# Autodesk Inventor assembly: XY Joint Left (Tulip)
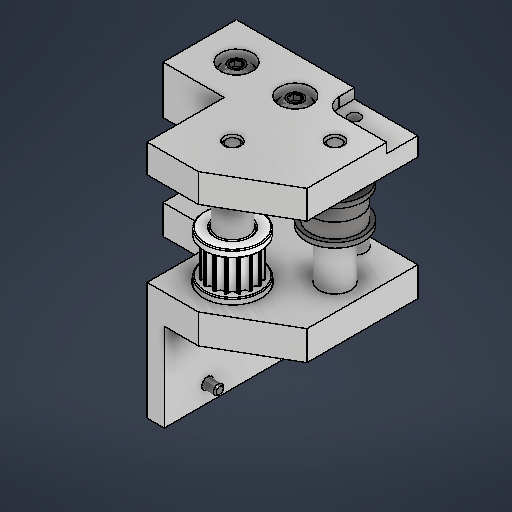
[picture p0: Inventor's stored thumbnail of the model, 512x512]
Saved by Autodesk Inventor 2026 (Build 300175050, 175E)
## iProperties
Created: 2025-05-24
Part Number: XY Joint Left (Tulip)
Document SubType Name: Assembly
Designer: Joshua Eah
Author: Joshua Eah
## Documents named in this file (14)
- C:\Users\Joshua Eah\Documents\GitHub\Voron-0\CAD\Tulip - Machined Parts\XY Joint Right\XY Joint Right Upper (Tulip).iam
- C:\Users\Joshua Eah\Documents\GitHub\Voron-0\CAD\Master Assembly\Hardware\f623-rs.ipt
- C:\Users\Joshua Eah\Documents\GitHub\Voron-0\CAD\Master Assembly\Hardware\M3_Washer.ipt
- C:\Users\Joshua Eah\Documents\GitHub\Voron-0\CAD\Tulip - Machined Parts\Spacers\Live Idler Spacer.ipt
- C:\Users\Joshua Eah\Documents\GitHub\Voron-0\CAD\Master Assembly\Hardware\3x30 Pin.ipt
- C:\Users\Joshua Eah\Documents\GitHub\Voron-0\CAD\Master Assembly\Hardware\F623 Stack.iam
- C:\Users\Joshua Eah\Documents\GitHub\Voron-0\CAD\Machined Parts\Spacers\Spacer.ipt
- C:\Users\Joshua Eah\Documents\GitHub\Voron-0\CAD\Tulip - Machined Parts\XY Joint Right\XY Joint Right Upper (Tulip).ipt
- C:\Users\Joshua Eah\Documents\GitHub\Voron-0\CAD\Tulip - Machined Parts\XY Joint Right\XY Joint Right Lower (Tulip).ipt
- C:\Users\Joshua Eah\Documents\GitHub\Voron-0\CAD\Master Assembly\Hardware\M3x6 BHCS.ipt
- C:\Users\Joshua Eah\Documents\GitHub\Voron-0\CAD\Master Assembly\Hardware\M3x12 BHCS.ipt
- C:\Users\Joshua Eah\Documents\GitHub\Voron-0\CAD\Master Assembly\Hardware\M2x6 FHCS.ipt
- C:\Users\Joshua Eah\Documents\GitHub\Voron-0\CAD\Tulip - Machined Parts\Spacers\Joint Spacer.ipt
- C:\Users\Joshua Eah\Documents\GitHub\Voron-0\CAD\Master Assembly\Hardware\16T_Pulley.ipt
## Components (21 placed, 13 different names)
1. XY Joint Right Upper (Tulip):1 — Insert:17, Insert:20, Insert:21, Insert:26, Mate:6
2. XY Joint Right Lower (Tulip):1 — Insert:16, Insert:19, Insert:22, Insert:23, Insert:24, Insert:25, Mate:8, Mate:10, Insert:28
3. f623-rs:1 — Insert:16, Mate:9
4. f623-rs:2 — Insert:4, Mate:5, Insert:17
5. M3_Washer:2 — Insert:4, Insert:14
6. Live Idler Spacer:1 — Insert:14, Insert:27
7. 16T_Pulley:1 — Insert:27
8. 3x30 Pin:1 — Mate:6, Flush:1, Mate:7, Mate:10
9. F623 Stack:1 [sub-assembly] — Insert:8, Insert:9
10. M3_Washer:3 — Insert:8
11. M3_Washer:4 — Insert:9, Insert:10
12. 3x30 Pin:2 — Mate:5, Flush:1, Mate:9
13. Spacer:1 — Insert:10, Mate:7, Mate:8
14. M3x6 BHCS:1 — Insert:19
15. M3x12 BHCS:1 — Insert:20
16. M3x12 BHCS:2 — Insert:21
17. M2x6 FHCS:1 — Insert:22
18. M2x6 FHCS:2 — Insert:23
19. M2x6 FHCS:3 — Insert:24
20. M2x6 FHCS:4 — Insert:25
21. Joint Spacer:1 — Insert:26, Insert:28
## Relationships (24: Insert 17, Mate 6, Flush 1)
- Insert:4: f623-rs:2 ↔ M3_Washer:2
- Mate:5: f623-rs:2 ↔ 3x30 Pin:2
- Insert:8: F623 Stack:1 ↔ M3_Washer:3
- Insert:9: F623 Stack:1 ↔ M3_Washer:4
- Insert:10: M3_Washer:4 ↔ Spacer:1
- Insert:14: M3_Washer:2 ↔ Live Idler Spacer:1
- Insert:16: XY Joint Right Lower (Tulip):1 ↔ f623-rs:1
- Insert:17: XY Joint Right Upper (Tulip):1 ↔ f623-rs:2
- Insert:19: XY Joint Right Lower (Tulip):1 ↔ M3x6 BHCS:1
- Insert:20: XY Joint Right Upper (Tulip):1 ↔ M3x12 BHCS:1
- Insert:21: XY Joint Right Upper (Tulip):1 ↔ M3x12 BHCS:2
- Insert:22: XY Joint Right Lower (Tulip):1 ↔ M2x6 FHCS:1
- Insert:23: XY Joint Right Lower (Tulip):1 ↔ M2x6 FHCS:2
- Insert:24: XY Joint Right Lower (Tulip):1 ↔ M2x6 FHCS:3
- Insert:25: XY Joint Right Lower (Tulip):1 ↔ M2x6 FHCS:4
- Insert:26: XY Joint Right Upper (Tulip):1 ↔ Joint Spacer:1
- Mate:6: XY Joint Right Upper (Tulip):1 ↔ 3x30 Pin:1
- Flush:1: 3x30 Pin:1 ↔ 3x30 Pin:2
- Mate:7: 3x30 Pin:1 ↔ Spacer:1
- Mate:8: XY Joint Right Lower (Tulip):1 ↔ Spacer:1
- Insert:27: Live Idler Spacer:1 ↔ 16T_Pulley:1
- Mate:9: f623-rs:1 ↔ 3x30 Pin:2
- Mate:10: XY Joint Right Lower (Tulip):1 ↔ 3x30 Pin:1
- Insert:28: XY Joint Right Lower (Tulip):1 ↔ Joint Spacer:1
